# Autodesk Inventor assembly: Gripper
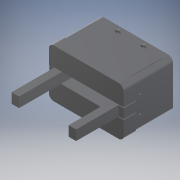
[picture p0: Inventor's stored thumbnail of the model, 180x180]
Saved by Autodesk Inventor 2017 (Build 210142000, 142)
## iProperties
Created: 2018-10-23
Part Number: Gripper
Document SubType Name: Assembly
Designer: Dell
Author: Dell
## Documents named in this file (6)
- C:\Users\Dell\Documents\GitHub\tr2\Gripper\Gripper.iam
- C:\Users\Dell\Documents\GitHub\tr2\Gripper\GA01.ipt
- C:\Users\Dell\Documents\GitHub\tr2\Gripper\AX-12A.ipt
- C:\Users\Dell\Documents\GitHub\tr2\Gripper\GA03.ipt
- C:\Users\Dell\Documents\GitHub\tr2\Gripper\Gripper\Design Accelerator\Spur Gears1.iam
- C:\Users\Dell\Documents\GitHub\tr2\Gripper\GA04.ipt
## Components (6 placed, 5 different names)
1. GA01:1 — Mate:8, Mate:9, Mate:12, Mate:22, Mate:23
2. GA03:1 — Mate:12, Mate:13, Mate:14, Mate:20
3. GA04:1 — Rotation/Translation:1, Flush:2, Mate:22
4. GA04:2 — Rotation/Translation:2, Flush:1, Mate:23
5. Spur Gears:1 [sub-assembly] — Mate:15, Mate:16, Rotation/Translation:1, Rotation/Translation:2, Flush:1, Flush:2
6. AX-12A:1 — Mate:8, Mate:9, Mate:13, Mate:14, Mate:15, Mate:16, Mate:20
## Relationships (14: Mate 10, RelateRotateTranslate 2, Flush 2)
- Mate:8: GA01:1 ↔ AX-12A:1
- Mate:9: GA01:1 ↔ AX-12A:1
- Mate:12: GA01:1 ↔ GA03:1
- Mate:13: GA03:1 ↔ AX-12A:1
- Mate:14: GA03:1 ↔ AX-12A:1
- Mate:15: Spur Gears:1 ↔ AX-12A:1
- Mate:16: Spur Gears:1 ↔ AX-12A:1
- Rotation/Translation:1 [RelateRotateTranslate] (131 mm): GA04:1 ↔ Spur Gears:1
- Rotation/Translation:2 [RelateRotateTranslate] (131 mm): GA04:2 ↔ Spur Gears:1
- Mate:20: GA03:1 ↔ AX-12A:1
- Flush:1: GA04:2 ↔ Spur Gears:1
- Flush:2: GA04:1 ↔ Spur Gears:1
- Mate:22: GA01:1 ↔ GA04:1
- Mate:23: GA01:1 ↔ GA04:2
